# Autodesk Inventor assembly: Structure
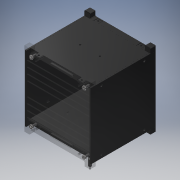
[picture p0: Inventor's stored thumbnail of the model, 180x180]
Saved by Autodesk Inventor 2018 (Build 220112000, 112)
## iProperties
Created: 2018-07-04
Part Number: Structure
Document SubType Name: Assembly
Designer: Bradley
Mass: 606.281 g
Surface Area: 1374.38 cm^2
Volume: 222.571 cm^3
Density: 2.72399 g/cm^3
Author: Bradley
## Documents named in this file (9)
- D:\Users\Bradley\Documents\CougsInSpace\CougSat1-Hardware\CougSat1-Structure\CADModel\Native\Structure.iam
- D:\Users\Bradley\Documents\CougsInSpace\CougSat1-Hardware\CougSat1-Structure\CADModel\Native\Structure_-Y.ipt
- D:\Users\Bradley\Documents\CougsInSpace\CougSat1-Hardware\CougSat1-Structure\CADModel\Native\Structure_+Y.ipt
- D:\Users\Bradley\Documents\CougsInSpace\CougSat1-Hardware\CougSat1-Structure\CADModel\Native\Structure_+Z.ipt
- D:\Users\Bradley\Documents\CougsInSpace\Resources\ComponentModels\Fasteners\Bolt_M3x0.35_12mm_SH.ipt
- D:\Users\Bradley\Documents\CougsInSpace\CougSat1-Hardware\CougSat1-Structure\CADModel\Native\Structure_-Z.ipt
- D:\Users\Bradley\Documents\CougsInSpace\CougSat1-Hardware\CougSat1-Structure\CADModel\Native\Structure_+X.ipt
- D:\Users\Bradley\Documents\CougsInSpace\CougSat1-Hardware\CougSat1-Structure\CADModel\Native\Structure_-X.ipt
- D:\Users\Bradley\Documents\CougsInSpace\Resources\ComponentModels\Hardware\Spring_Separation.ipt
## Components (16 placed, 8 different names)
1. Structure_-Y:1 — Flush:1, Flush:2, Insert:1, Insert:2, Insert:3, Insert:4, Insert:9, Insert:10, Insert:14, Insert:15, Insert:21
2. Structure_+Y:1 — Flush:3, Flush:4, Insert:5, Insert:6, Insert:7, Insert:8, Insert:11, Insert:12, Insert:13, Insert:22
3. Structure_+Z:1 — Insert:9, Insert:10, Insert:11, Insert:12, Flush:5, Mate:1, Insert:16, Insert:17, Insert:18
4. Bolt_M3x0.35_12mm_SH:1 — Insert:1
5. Bolt_M3x0.35_12mm_SH:2 — Insert:2
6. Bolt_M3x0.35_12mm_SH:3 — Insert:3
7. Bolt_M3x0.35_12mm_SH:4 — Insert:4
8. Bolt_M3x0.35_12mm_SH:5 — Insert:5
9. Bolt_M3x0.35_12mm_SH:6 — Insert:7
10. Bolt_M3x0.35_12mm_SH:7 — Insert:6
11. Bolt_M3x0.35_12mm_SH:8 — Insert:8
12. Structure_-Z:1 — Insert:13, Insert:14, Insert:15, Insert:19, Insert:20
13. Structure_+X:1 — Mate:1, Flush:6, Flush:7, Insert:16, Insert:19
14. Structure_-X:1 — Insert:17, Insert:18, Insert:20
15. Spring_Separation:1 — Insert:22
16. Spring_Separation:2 — Insert:21
## Relationships (30: Insert 22, Flush 7, Mate 1)
- Flush:1: Structure_-Y:1
- Flush:2: Structure_-Y:1
- Flush:3: Structure_+Y:1
- Flush:4: Structure_+Y:1
- Insert:1: Structure_-Y:1 ↔ Bolt_M3x0.35_12mm_SH:1
- Insert:2: Structure_-Y:1 ↔ Bolt_M3x0.35_12mm_SH:2
- Insert:3: Structure_-Y:1 ↔ Bolt_M3x0.35_12mm_SH:3
- Insert:4: Structure_-Y:1 ↔ Bolt_M3x0.35_12mm_SH:4
- Insert:5: Structure_+Y:1 ↔ Bolt_M3x0.35_12mm_SH:5
- Insert:6: Structure_+Y:1 ↔ Bolt_M3x0.35_12mm_SH:7
- Insert:7: Structure_+Y:1 ↔ Bolt_M3x0.35_12mm_SH:6
- Insert:8: Structure_+Y:1 ↔ Bolt_M3x0.35_12mm_SH:8
- Insert:9: Structure_-Y:1 ↔ Structure_+Z:1
- Insert:10: Structure_-Y:1 ↔ Structure_+Z:1
- Insert:11: Structure_+Y:1 ↔ Structure_+Z:1
- Insert:12: Structure_+Y:1 ↔ Structure_+Z:1
- Flush:5: Structure_+Z:1
- Insert:13: Structure_+Y:1 ↔ Structure_-Z:1
- Insert:14: Structure_-Y:1 ↔ Structure_-Z:1
- Insert:15: Structure_-Y:1 ↔ Structure_-Z:1
- Mate:1: Structure_+Z:1 ↔ Structure_+X:1
- Flush:6: Structure_+X:1
- Flush:7: Structure_+X:1
- Insert:16: Structure_+Z:1 ↔ Structure_+X:1
- Insert:17: Structure_+Z:1 ↔ Structure_-X:1
- Insert:18: Structure_+Z:1 ↔ Structure_-X:1
- Insert:19: Structure_-Z:1 ↔ Structure_+X:1
- Insert:20: Structure_-Z:1 ↔ Structure_-X:1
- Insert:21: Structure_-Y:1 ↔ Spring_Separation:2
- Insert:22: Structure_+Y:1 ↔ Spring_Separation:1
